# Autodesk Inventor assembly: Bunnybot
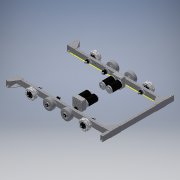
[picture p0: Inventor's stored thumbnail of the model, 180x180]
Saved by Autodesk Inventor 2018 (Build 220112000, 112)
## iProperties
Created: 2018-09-05
Part Number: Bunnybot
Document SubType Name: Assembly
Designer: baoan
Author: baoan
## Documents named in this file (16)
- C:\Users\baoan\Documents\Inventor\Bunnybots\Drivetrain\Drivetrain.iam
- C:\Users\baoan\Documents\Inventor\Bunnybots\Drivetrain\Drivetrain_length.ipt
- C:\Users\baoan\Documents\Inventor\Bunnybots\Drivetrain\Drivetrain_width.ipt
- C:\Users\baoan\Documents\Inventor\Bunnybots\Drivetrain\Center Bearing Block.ipt
- C:\Users\baoan\Documents\Inventor\Bunnybots\Drivetrain\WCP_Side_Bearing_Block_Kit_217-3436.iam
- C:\Users\baoan\Documents\Inventor\Bunnybots\Drivetrain\Drivetrain_hex_shaft.ipt
- C:\Users\baoan\Documents\Inventor\Bunnybots\Drivetrain\4_Omni-Directional_Wheel_v2_276-6194.iam
- C:\Users\baoan\Documents\Inventor\Bunnybots\Drivetrain\Hole_to_hex.ipt
- C:\Users\baoan\Documents\Inventor\Bunnybots\Drivetrain\Bearing.ipt
- C:\Users\baoan\Documents\Inventor\Bunnybots\Drivetrain\Shaft_collar.ipt
- C:\Users\baoan\Documents\Inventor\Bunnybots\Drivetrain\Drivetrain_sprockets.ipt
- C:\Users\baoan\Documents\Inventor\Bunnybots\Drivetrain\Colson_wheel.ipt
- C:\Users\baoan\Documents\Inventor\Bunnybots\Cimscellaneous\217-2454-STEP-Rev2.iam
- C:\Users\baoan\Documents\Inventor\Bunnybots\Drivetrain\Gearbox_hex_shaft.ipt
- C:\Users\baoan\Documents\Inventor\Bunnybots\Drivetrain\Drivetrain_gussets.ipt
- C:\Users\baoan\Documents\Inventor\Bunnybots\Drivetrain\Drivetrain_short_front.ipt
## Components (83 placed, 15 different names)
1. Drivetrain_width:1 — Flush:10, Flush:18, Flush:33, Mate:187, Mate:188, Flush:34, Flush:36, Mate:191, Flush:42, Flush:44, Mate:194, Flush:51, Flush:52, Flush:54
2. Drivetrain_length:3 — Angle:1, Mate:159, Flush:41, Mate:192, Flush:43, Flush:48, Mate:193, Mate:194, Flush:49, Flush:50, Flush:51, Flush:52, Mate:197, Flush:58, Flush:59
3. Center Bearing Block:2 — Insert:2
4. WCP_Side_Bearing_Block_Kit_217-3436:4 [sub-assembly] — Insert:3, Insert:5
5. WCP_Side_Bearing_Block_Kit_217-3436:5 [sub-assembly] — Insert:4, Insert:6
6. WCP_Side_Bearing_Block_Kit_217-3436:6 [sub-assembly] — Mate:38, Insert:1, Mate:39
7. Drivetrain_hex_shaft:6 — Mate:40, Mate:41, Mate:48, Mate:49, Mate:50, Mate:51, Mate:53, Mate:54, Mate:70, Mate:71, Flush:10, Flush:11
8. 4_Omni-Directional_Wheel_v2_276-6194:1 [sub-assembly] — Mate:32, Mate:33, Mate:34, Mate:35, Mate:36, Mate:37
9. Hole_to_hex:1 — Mate:32, Mate:33, Mate:34, Mate:49
10. Hole_to_hex:2 — Mate:35, Mate:36, Mate:37, Mate:48, Mate:52
11. Bearing:1 — Mate:38, Mate:39, Mate:40, Mate:41
12. Bearing:2 — Insert:1, Mate:185
13. Bearing:3 — Insert:2, Mate:100, Mate:101
14. Bearing:4 — Insert:3, Mate:68, Mate:69
15. Bearing:5 — Insert:4
16. Bearing:6 — Insert:5
17. Bearing:7 — Insert:6, Mate:90, Mate:91
18. Shaft_collar:1 — Mate:50, Mate:51, Mate:52, Flush:11
19. Drivetrain_sprockets:1 — Mate:53, Mate:54
20. Drivetrain_hex_shaft:7 — Mate:68, Mate:69, Flush:8, Mate:72, Mate:73
21. 4_Omni-Directional_Wheel_v2_276-6194:2 [sub-assembly] — Flush:13
22. Hole_to_hex:3
23. Hole_to_hex:4
24. Shaft_collar:2 — Flush:8
25. Drivetrain_sprockets:2
26. Drivetrain_sprockets:3 — Mate:70, Mate:71, Flush:31, Mate:185
27. Drivetrain_sprockets:4 — Mate:72, Mate:73, Flush:14
28. Colson_wheel:1 — Mate:87, Mate:88, Mate:89, Flush:13
29. Drivetrain_hex_shaft:8 — Mate:87, Mate:88, Mate:90, Mate:91, Mate:92, Mate:93, Mate:94, Mate:95
30. Shaft_collar:3 — Mate:89
31. Drivetrain_sprockets:5 — Mate:92, Mate:93, Mate:96, Flush:14, Flush:30
32. Drivetrain_sprockets:6 — Mate:94, Mate:95, Mate:96
33. 217-2454-STEP-Rev2:1 [sub-assembly] — Mate:97, Mate:98, Mate:99, Angle:1, Mate:159
34. Gearbox_hex_shaft:1 — Mate:97, Mate:98, Mate:99, Mate:100, Mate:101, Mate:160, Mate:161, Mate:162, Mate:163, Flush:23, Mate:167, Mate:168
35. Drivetrain_length:4 — Insert:13, Mate:183, Angle:2, Mate:186, Flush:32, Mate:187, Flush:35, Flush:36, Flush:46, Mate:195, Flush:53, Flush:54, Flush:55, Mate:199, Flush:62
36. WCP_Side_Bearing_Block_Kit_217-3436:7 [sub-assembly]
37. WCP_Side_Bearing_Block_Kit_217-3436:8 [sub-assembly]
38. WCP_Side_Bearing_Block_Kit_217-3436:9 [sub-assembly]
39. Bearing:8 — Mate:184
40. Bearing:9 — Mate:130, Mate:131
41. Bearing:11
42. Bearing:12 — Mate:157, Mate:158
43. Bearing:13 — Mate:145, Mate:146
44. Bearing:14
45. Center Bearing Block:3 — Insert:13, Insert:14
46. Bearing:15 — Insert:14, Mate:181, Mate:182
47. Drivetrain_hex_shaft:9 — Mate:130, Mate:131, Flush:18
48. 4_Omni-Directional_Wheel_v2_276-6194:3 [sub-assembly]
49. Hole_to_hex:5
50. Hole_to_hex:6
51. Shaft_collar:4
52. Drivetrain_sprockets:7 — Flush:29, Mate:184
53. Drivetrain_hex_shaft:10 — Mate:145, Mate:146
54. 4_Omni-Directional_Wheel_v2_276-6194:4 [sub-assembly] — Flush:22
55. Hole_to_hex:7
56. Hole_to_hex:8
57. Shaft_collar:5
58. Drivetrain_sprockets:8 — Flush:28
59. Colson_wheel:2 — Flush:22
60. Drivetrain_hex_shaft:11 — Mate:157, Mate:158
61. Shaft_collar:6
62. Drivetrain_sprockets:9 — Flush:27, Flush:28
63. Drivetrain_sprockets:10
64. Colson_wheel:3 — Mate:160, Mate:161, Mate:164
65. Shaft_collar:7 — Mate:162, Mate:163, Flush:23, Mate:164
66. Drivetrain_sprockets:11 — Mate:166, Flush:24, Mate:167, Mate:168, Flush:30, Flush:31
67. Drivetrain_sprockets:12 — Mate:166, Flush:24
68. 217-2454-STEP-Rev2:2 [sub-assembly] — Mate:183, Angle:2
69. Gearbox_hex_shaft:2 — Mate:181, Mate:182
70. Colson_wheel:4
71. Shaft_collar:8
72. Drivetrain_sprockets:13 — Flush:27, Flush:29
73. Drivetrain_sprockets:14
74. Drivetrain_gussets:1 — Mate:186, Flush:32, Flush:33
75. Drivetrain_gussets:2 — Mate:188, Flush:34, Flush:35
76. Drivetrain_gussets:5 — Mate:191, Flush:41, Flush:42
77. Drivetrain_gussets:6 — Mate:192, Flush:43, Flush:44
78. Drivetrain_gussets:7 — Flush:46, Mate:196, Flush:56
79. Drivetrain_gussets:8 — Flush:48, Mate:197, Flush:57, Flush:58
80. Drivetrain_short_front:1 — Mate:193, Flush:49, Flush:50, Flush:57, Mate:198, Flush:60
81. Drivetrain_short_front:2 — Mate:195, Flush:53, Mate:196, Flush:55, Flush:56, Flush:61
82. Drivetrain_gussets:9 — Mate:198, Flush:59, Flush:60
83. Drivetrain_gussets:10 — Mate:199, Flush:61, Flush:62
## Relationships (217: Mate 157, Flush 45, Insert 13, Angle 2)
- [Mate]: Drivetrain_length:3 ↔ Center Bearing Block:2
- [Mate]: Drivetrain_length:3 ↔ Center Bearing Block:2
- [Mate]: Drivetrain_length:3 ↔ Center Bearing Block:2
- [Mate]: Drivetrain_length:3 ↔ WCP_Side_Bearing_Block_Kit_217-3436:4
- [Mate]: Drivetrain_length:3 ↔ WCP_Side_Bearing_Block_Kit_217-3436:4
- [Mate]: Drivetrain_length:3 ↔ WCP_Side_Bearing_Block_Kit_217-3436:4
- [Mate]: Drivetrain_length:3 ↔ WCP_Side_Bearing_Block_Kit_217-3436:5
- [Mate]: Drivetrain_length:3 ↔ WCP_Side_Bearing_Block_Kit_217-3436:5
- [Mate]: Drivetrain_length:3 ↔ WCP_Side_Bearing_Block_Kit_217-3436:5
- [Mate]: Drivetrain_length:3 ↔ WCP_Side_Bearing_Block_Kit_217-3436:6
- [Mate]: Drivetrain_length:3 ↔ WCP_Side_Bearing_Block_Kit_217-3436:6
- [Mate]: Drivetrain_length:3 ↔ WCP_Side_Bearing_Block_Kit_217-3436:6
- Mate:32: 4_Omni-Directional_Wheel_v2_276-6194:1 ↔ Hole_to_hex:1
- Mate:33: 4_Omni-Directional_Wheel_v2_276-6194:1 ↔ Hole_to_hex:1
- Mate:34: 4_Omni-Directional_Wheel_v2_276-6194:1 ↔ Hole_to_hex:1
- Mate:35: 4_Omni-Directional_Wheel_v2_276-6194:1 ↔ Hole_to_hex:2
- Mate:36: 4_Omni-Directional_Wheel_v2_276-6194:1 ↔ Hole_to_hex:2
- Mate:37: 4_Omni-Directional_Wheel_v2_276-6194:1 ↔ Hole_to_hex:2
- Mate:38: WCP_Side_Bearing_Block_Kit_217-3436:6 ↔ Bearing:1
- Insert:1: WCP_Side_Bearing_Block_Kit_217-3436:6 ↔ Bearing:2
- Mate:39: WCP_Side_Bearing_Block_Kit_217-3436:6 ↔ Bearing:1
- Insert:2: Center Bearing Block:2 ↔ Bearing:3
- Insert:3: WCP_Side_Bearing_Block_Kit_217-3436:4 ↔ Bearing:4
- Insert:4: WCP_Side_Bearing_Block_Kit_217-3436:5 ↔ Bearing:5
- Insert:5: WCP_Side_Bearing_Block_Kit_217-3436:4 ↔ Bearing:6
- Insert:6: WCP_Side_Bearing_Block_Kit_217-3436:5 ↔ Bearing:7
- Mate:40: Drivetrain_hex_shaft:6 ↔ Bearing:1
- Mate:41: Drivetrain_hex_shaft:6 ↔ Bearing:1
- Mate:48: Drivetrain_hex_shaft:6 ↔ Hole_to_hex:2
- Mate:49: Drivetrain_hex_shaft:6 ↔ Hole_to_hex:1
- Mate:50: Drivetrain_hex_shaft:6 ↔ Shaft_collar:1
- Mate:51: Drivetrain_hex_shaft:6 ↔ Shaft_collar:1
- Mate:52: Hole_to_hex:2 ↔ Shaft_collar:1
- Mate:53: Drivetrain_hex_shaft:6 ↔ Drivetrain_sprockets:1
- Mate:54: Drivetrain_hex_shaft:6 ↔ Drivetrain_sprockets:1
- [Mate]: 4_Omni-Directional_Wheel_v2_276-6194:2 ↔ Hole_to_hex:3
- [Mate]: 4_Omni-Directional_Wheel_v2_276-6194:2 ↔ Hole_to_hex:3
- [Mate]: 4_Omni-Directional_Wheel_v2_276-6194:2 ↔ Hole_to_hex:3
- [Mate]: 4_Omni-Directional_Wheel_v2_276-6194:2 ↔ Hole_to_hex:4
- [Mate]: 4_Omni-Directional_Wheel_v2_276-6194:2 ↔ Hole_to_hex:4
- [Mate]: 4_Omni-Directional_Wheel_v2_276-6194:2 ↔ Hole_to_hex:4
- [Mate]: Drivetrain_hex_shaft:7 ↔ Hole_to_hex:4
- [Mate]: Drivetrain_hex_shaft:7 ↔ Hole_to_hex:3
- [Mate]: Drivetrain_hex_shaft:7 ↔ Shaft_collar:2
- [Mate]: Drivetrain_hex_shaft:7 ↔ Shaft_collar:2
- [Mate]: Hole_to_hex:4 ↔ Shaft_collar:2
- [Mate]: Drivetrain_hex_shaft:7 ↔ Drivetrain_sprockets:2
- [Mate]: Drivetrain_hex_shaft:7 ↔ Drivetrain_sprockets:2
- Mate:68: Bearing:4 ↔ Drivetrain_hex_shaft:7
- Mate:69: Bearing:4 ↔ Drivetrain_hex_shaft:7
- Flush:8 (-3.175 mm): Drivetrain_hex_shaft:7 ↔ Shaft_collar:2
- Mate:70: Drivetrain_hex_shaft:6 ↔ Drivetrain_sprockets:3
- Mate:71: Drivetrain_hex_shaft:6 ↔ Drivetrain_sprockets:3
- Flush:10: Drivetrain_width:1 ↔ Drivetrain_hex_shaft:6
- Flush:11 (-3.175 mm): Drivetrain_hex_shaft:6 ↔ Shaft_collar:1
- Mate:72: Drivetrain_hex_shaft:7 ↔ Drivetrain_sprockets:4
- Mate:73: Drivetrain_hex_shaft:7 ↔ Drivetrain_sprockets:4
- [Mate]: Drivetrain_hex_shaft:8 ↔ Shaft_collar:3
- [Mate]: Drivetrain_hex_shaft:8 ↔ Shaft_collar:3
- [Flush] (-3.175 mm): Drivetrain_hex_shaft:8 ↔ Shaft_collar:3
- Mate:87: Colson_wheel:1 ↔ Drivetrain_hex_shaft:8
- Mate:88: Colson_wheel:1 ↔ Drivetrain_hex_shaft:8
- Mate:89: Colson_wheel:1 ↔ Shaft_collar:3
- Mate:90: Bearing:7 ↔ Drivetrain_hex_shaft:8
- Mate:91: Bearing:7 ↔ Drivetrain_hex_shaft:8
- Flush:13: 4_Omni-Directional_Wheel_v2_276-6194:2 ↔ Colson_wheel:1
- Mate:92: Drivetrain_hex_shaft:8 ↔ Drivetrain_sprockets:5
- Mate:93: Drivetrain_hex_shaft:8 ↔ Drivetrain_sprockets:5
- Mate:94: Drivetrain_hex_shaft:8 ↔ Drivetrain_sprockets:6
- Mate:95: Drivetrain_hex_shaft:8 ↔ Drivetrain_sprockets:6
- Mate:96: Drivetrain_sprockets:5 ↔ Drivetrain_sprockets:6
- Flush:14: Drivetrain_sprockets:4 ↔ Drivetrain_sprockets:5
- Mate:97: 217-2454-STEP-Rev2:1 ↔ Gearbox_hex_shaft:1
- Mate:98: 217-2454-STEP-Rev2:1 ↔ Gearbox_hex_shaft:1
- Mate:99: 217-2454-STEP-Rev2:1 ↔ Gearbox_hex_shaft:1
- Mate:100: Bearing:3 ↔ Gearbox_hex_shaft:1
- Mate:101: Bearing:3 ↔ Gearbox_hex_shaft:1
- Angle:1 (0 deg): Drivetrain_length:3 ↔ 217-2454-STEP-Rev2:1
- [Mate]: Drivetrain_length:4 ↔ WCP_Side_Bearing_Block_Kit_217-3436:7
- [Mate]: Drivetrain_length:4 ↔ WCP_Side_Bearing_Block_Kit_217-3436:7
- [Mate]: Drivetrain_length:4 ↔ WCP_Side_Bearing_Block_Kit_217-3436:7
- [Mate]: Drivetrain_length:4 ↔ WCP_Side_Bearing_Block_Kit_217-3436:8
- [Mate]: Drivetrain_length:4 ↔ WCP_Side_Bearing_Block_Kit_217-3436:8
- [Mate]: Drivetrain_length:4 ↔ WCP_Side_Bearing_Block_Kit_217-3436:8
- [Mate]: Drivetrain_length:4 ↔ WCP_Side_Bearing_Block_Kit_217-3436:9
- [Mate]: Drivetrain_length:4 ↔ WCP_Side_Bearing_Block_Kit_217-3436:9
- [Mate]: Drivetrain_length:4 ↔ WCP_Side_Bearing_Block_Kit_217-3436:9
- [Mate]: WCP_Side_Bearing_Block_Kit_217-3436:9 ↔ Bearing:8
- [Insert]: WCP_Side_Bearing_Block_Kit_217-3436:9 ↔ Bearing:9
- [Mate]: WCP_Side_Bearing_Block_Kit_217-3436:9 ↔ Bearing:8
- [Insert]: WCP_Side_Bearing_Block_Kit_217-3436:7 ↔ Bearing:11
- [Insert]: WCP_Side_Bearing_Block_Kit_217-3436:8 ↔ Bearing:12
- [Insert]: WCP_Side_Bearing_Block_Kit_217-3436:7 ↔ Bearing:13
- [Insert]: WCP_Side_Bearing_Block_Kit_217-3436:8 ↔ Bearing:14
- Insert:13: Drivetrain_length:4 ↔ Center Bearing Block:3
- Insert:14: Center Bearing Block:3 ↔ Bearing:15
- [Mate]: 4_Omni-Directional_Wheel_v2_276-6194:3 ↔ Hole_to_hex:5
- [Mate]: 4_Omni-Directional_Wheel_v2_276-6194:3 ↔ Hole_to_hex:5
- [Mate]: 4_Omni-Directional_Wheel_v2_276-6194:3 ↔ Hole_to_hex:5
- [Mate]: 4_Omni-Directional_Wheel_v2_276-6194:3 ↔ Hole_to_hex:6
- [Mate]: 4_Omni-Directional_Wheel_v2_276-6194:3 ↔ Hole_to_hex:6
- [Mate]: 4_Omni-Directional_Wheel_v2_276-6194:3 ↔ Hole_to_hex:6
- [Mate]: Drivetrain_hex_shaft:9 ↔ Hole_to_hex:6
- [Mate]: Drivetrain_hex_shaft:9 ↔ Hole_to_hex:5
- [Mate]: Drivetrain_hex_shaft:9 ↔ Shaft_collar:4
- [Mate]: Drivetrain_hex_shaft:9 ↔ Shaft_collar:4
- [Mate]: Hole_to_hex:6 ↔ Shaft_collar:4
- [Mate]: Drivetrain_hex_shaft:9 ↔ Drivetrain_sprockets:7
- [Mate]: Drivetrain_hex_shaft:9 ↔ Drivetrain_sprockets:7
- [Flush] (-3.175 mm): Drivetrain_hex_shaft:9 ↔ Shaft_collar:4
- Mate:130: Bearing:9 ↔ Drivetrain_hex_shaft:9
- Mate:131: Bearing:9 ↔ Drivetrain_hex_shaft:9
- Flush:18: Drivetrain_width:1 ↔ Drivetrain_hex_shaft:9
- [Mate]: 4_Omni-Directional_Wheel_v2_276-6194:4 ↔ Hole_to_hex:7
- [Mate]: 4_Omni-Directional_Wheel_v2_276-6194:4 ↔ Hole_to_hex:7
- [Mate]: 4_Omni-Directional_Wheel_v2_276-6194:4 ↔ Hole_to_hex:7
- [Mate]: 4_Omni-Directional_Wheel_v2_276-6194:4 ↔ Hole_to_hex:8
- [Mate]: 4_Omni-Directional_Wheel_v2_276-6194:4 ↔ Hole_to_hex:8
- [Mate]: 4_Omni-Directional_Wheel_v2_276-6194:4 ↔ Hole_to_hex:8
- [Mate]: Drivetrain_hex_shaft:10 ↔ Hole_to_hex:8
- [Mate]: Drivetrain_hex_shaft:10 ↔ Hole_to_hex:7
- [Mate]: Drivetrain_hex_shaft:10 ↔ Shaft_collar:5
- [Mate]: Drivetrain_hex_shaft:10 ↔ Shaft_collar:5
- [Mate]: Hole_to_hex:8 ↔ Shaft_collar:5
- [Mate]: Drivetrain_hex_shaft:10 ↔ Drivetrain_sprockets:8
- [Mate]: Drivetrain_hex_shaft:10 ↔ Drivetrain_sprockets:8
- [Flush] (-3.175 mm): Drivetrain_hex_shaft:10 ↔ Shaft_collar:5
- Mate:145: Bearing:13 ↔ Drivetrain_hex_shaft:10
- Mate:146: Bearing:13 ↔ Drivetrain_hex_shaft:10
- [Mate]: Drivetrain_hex_shaft:11 ↔ Shaft_collar:6
- [Mate]: Drivetrain_hex_shaft:11 ↔ Shaft_collar:6
- [Flush] (-3.175 mm): Drivetrain_hex_shaft:11 ↔ Shaft_collar:6
- [Mate]: Colson_wheel:2 ↔ Drivetrain_hex_shaft:11
- [Mate]: Colson_wheel:2 ↔ Drivetrain_hex_shaft:11
- [Mate]: Colson_wheel:2 ↔ Shaft_collar:6
- [Mate]: Drivetrain_hex_shaft:11 ↔ Drivetrain_sprockets:9
- [Mate]: Drivetrain_hex_shaft:11 ↔ Drivetrain_sprockets:9
- [Mate]: Drivetrain_hex_shaft:11 ↔ Drivetrain_sprockets:10
- [Mate]: Drivetrain_hex_shaft:11 ↔ Drivetrain_sprockets:10
- [Mate]: Drivetrain_sprockets:9 ↔ Drivetrain_sprockets:10
- Mate:157: Bearing:12 ↔ Drivetrain_hex_shaft:11
- Mate:158: Bearing:12 ↔ Drivetrain_hex_shaft:11
- Flush:22: 4_Omni-Directional_Wheel_v2_276-6194:4 ↔ Colson_wheel:2
- Mate:159 (38.1 mm): Drivetrain_length:3 ↔ 217-2454-STEP-Rev2:1
- Mate:160: Gearbox_hex_shaft:1 ↔ Colson_wheel:3
- Mate:161: Gearbox_hex_shaft:1 ↔ Colson_wheel:3
- Mate:162: Gearbox_hex_shaft:1 ↔ Shaft_collar:7
- Mate:163: Gearbox_hex_shaft:1 ↔ Shaft_collar:7
- Flush:23 (-3.175 mm): Gearbox_hex_shaft:1 ↔ Shaft_collar:7
- Mate:164: Colson_wheel:3 ↔ Shaft_collar:7
- [Mate]: Drivetrain_sprockets:11 ↔ Drivetrain_sprockets:12
- Mate:166: Drivetrain_sprockets:11 ↔ Drivetrain_sprockets:12
- Flush:24: Drivetrain_sprockets:11 ↔ Drivetrain_sprockets:12
- Mate:167: Gearbox_hex_shaft:1 ↔ Drivetrain_sprockets:11
- Mate:168: Gearbox_hex_shaft:1 ↔ Drivetrain_sprockets:11
- [Mate]: 217-2454-STEP-Rev2:2 ↔ Gearbox_hex_shaft:2
- [Mate]: 217-2454-STEP-Rev2:2 ↔ Gearbox_hex_shaft:2
- [Mate]: 217-2454-STEP-Rev2:2 ↔ Gearbox_hex_shaft:2
- [Mate]: Gearbox_hex_shaft:2 ↔ Colson_wheel:4
- [Mate]: Gearbox_hex_shaft:2 ↔ Colson_wheel:4
- [Mate]: Gearbox_hex_shaft:2 ↔ Shaft_collar:8
- [Mate]: Gearbox_hex_shaft:2 ↔ Shaft_collar:8
- [Flush] (-3.175 mm): Gearbox_hex_shaft:2 ↔ Shaft_collar:8
- [Mate]: Colson_wheel:4 ↔ Shaft_collar:8
- [Mate]: Drivetrain_sprockets:13 ↔ Drivetrain_sprockets:14
- [Mate]: Drivetrain_sprockets:13 ↔ Drivetrain_sprockets:14
- [Flush]: Drivetrain_sprockets:13 ↔ Drivetrain_sprockets:14
- [Mate]: Gearbox_hex_shaft:2 ↔ Drivetrain_sprockets:13
- [Mate]: Gearbox_hex_shaft:2 ↔ Drivetrain_sprockets:13
- Mate:181: Bearing:15 ↔ Gearbox_hex_shaft:2
- Mate:182: Bearing:15 ↔ Gearbox_hex_shaft:2
- Mate:183 (38.1 mm): Drivetrain_length:4 ↔ 217-2454-STEP-Rev2:2
- Flush:27: Drivetrain_sprockets:9 ↔ Drivetrain_sprockets:13
- Flush:28: Drivetrain_sprockets:8 ↔ Drivetrain_sprockets:9
- Flush:29: Drivetrain_sprockets:7 ↔ Drivetrain_sprockets:13
- Flush:30: Drivetrain_sprockets:5 ↔ Drivetrain_sprockets:11
- Flush:31: Drivetrain_sprockets:3 ↔ Drivetrain_sprockets:11
- Mate:184 (8.255 mm): Bearing:8 ↔ Drivetrain_sprockets:7
- Mate:185 (8.255 mm): Bearing:2 ↔ Drivetrain_sprockets:3
- Angle:2 (0 deg): Drivetrain_length:4 ↔ 217-2454-STEP-Rev2:2
- Mate:186: Drivetrain_length:4 ↔ Drivetrain_gussets:1
- Flush:32: Drivetrain_length:4 ↔ Drivetrain_gussets:1
- Flush:33: Drivetrain_width:1 ↔ Drivetrain_gussets:1
- Mate:187: Drivetrain_width:1 ↔ Drivetrain_length:4
- Mate:188: Drivetrain_width:1 ↔ Drivetrain_gussets:2
- Flush:34: Drivetrain_width:1 ↔ Drivetrain_gussets:2
- Flush:35: Drivetrain_length:4 ↔ Drivetrain_gussets:2
- Flush:36: Drivetrain_width:1 ↔ Drivetrain_length:4
- Mate:191: Drivetrain_width:1 ↔ Drivetrain_gussets:5
- Flush:41: Drivetrain_length:3 ↔ Drivetrain_gussets:5
- Flush:42: Drivetrain_width:1 ↔ Drivetrain_gussets:5
- Mate:192: Drivetrain_length:3 ↔ Drivetrain_gussets:6
- Flush:43: Drivetrain_length:3 ↔ Drivetrain_gussets:6
- Flush:44: Drivetrain_width:1 ↔ Drivetrain_gussets:6
- Flush:46: Drivetrain_length:4 ↔ Drivetrain_gussets:7
- Flush:48: Drivetrain_length:3 ↔ Drivetrain_gussets:8
- Mate:193: Drivetrain_length:3 ↔ Drivetrain_short_front:1
- Mate:194: Drivetrain_width:1 ↔ Drivetrain_length:3
- Flush:49: Drivetrain_length:3 ↔ Drivetrain_short_front:1
- Flush:50: Drivetrain_length:3 ↔ Drivetrain_short_front:1
- Flush:51 (76.2 mm): Drivetrain_width:1 ↔ Drivetrain_length:3
- Flush:52: Drivetrain_width:1 ↔ Drivetrain_length:3
- Mate:195: Drivetrain_length:4 ↔ Drivetrain_short_front:2
- Flush:53: Drivetrain_length:4 ↔ Drivetrain_short_front:2
- Mate:196: Drivetrain_gussets:7 ↔ Drivetrain_short_front:2
- Flush:54 (76.2 mm): Drivetrain_width:1 ↔ Drivetrain_length:4
- Flush:55: Drivetrain_length:4 ↔ Drivetrain_short_front:2
- Flush:56: Drivetrain_gussets:7 ↔ Drivetrain_short_front:2
- Mate:197: Drivetrain_length:3 ↔ Drivetrain_gussets:8
- Flush:57: Drivetrain_gussets:8 ↔ Drivetrain_short_front:1
- Flush:58: Drivetrain_length:3 ↔ Drivetrain_gussets:8
- Mate:198: Drivetrain_short_front:1 ↔ Drivetrain_gussets:9
- Flush:59: Drivetrain_length:3 ↔ Drivetrain_gussets:9
- Flush:60: Drivetrain_short_front:1 ↔ Drivetrain_gussets:9
- Mate:199: Drivetrain_length:4 ↔ Drivetrain_gussets:10
- Flush:61: Drivetrain_short_front:2 ↔ Drivetrain_gussets:10
- Flush:62: Drivetrain_length:4 ↔ Drivetrain_gussets:10
## Named parameters: d33_d18 = 0 mm, d34_d19 = 0 mm, d35_d22 = 0 mm, d36_d24 = 0 mm, d37_d25 = 0 mm, d38_d26 = 0 mm, d39_d27 = 0 mm, d40_d28 = 0 mm, d41_d29 = 0 mm, d42_d30 = 0 mm, d43_d31 = 0 mm, d44_d32 = 0 mm, d78_d71 = 0 mm, d79_d72 = 0 mm, d80_d73 = 0 mm, d81_d74 = 0 mm, d82_d75 = 0 mm, d83_d76 = 0 mm, d84_d77 = 0 mm, d85_d48 = 0 mm, d86_d49 = 0 mm, d87_d50 = 0 mm, d88_d51 = 0 mm, d89_d52 = 0 mm, d90_d53 = 0 mm, d105_d80_d73 = 0 mm, d106_d81_d74 = 0 mm, d114_d93 = -3.175 mm, d139_d36_d24 = 0 mm, d140_d37_d25 = 0 mm, d141_d38_d26 = 0 mm, d142_d39_d27 = 0 mm, d143_d40_d28 = 0 mm, d144_d41_d29 = 0 mm, d145_d42_d30 = 0 mm, d146_d43_d31 = 0 mm, d147_d44_d32 = 0 mm, d148_d54 = 0 mm, d149_d56 = 0 mm, d150_d57 = 0 mm, d152_d59 = 0 mm, d153_d60 = 0 mm, d154_d61 = 0 mm, d155_d62 = 0 mm, d161_d98 = -3.175 mm, d162_d71 = 0 mm, d163_d72 = 0 mm, d164_d73 = 0 mm, d165_d74 = 0 mm, d166_d75 = 0 mm, d167_d95 = 0 mm, d168_d96 = 0 mm, d169_d48 = 0 mm, d170_d49 = 0 mm, d171_d50 = 0 mm, d172_d51 = 0 mm, d173_d52 = 0 mm, d174_d53 = 0 mm, d178_d161_d98 = -3.175 mm, d179_d162_d71 = 0 mm, d180_d163_d72 = 0 mm, d181_d164_d73 = 0 mm, d182_d165_d74 = 0 mm, d183_d166_d75 = 0 mm, d184_d167_d95 = 0 mm, d185_d168_d96 = 0 mm, d186_d169_d48 = 0 mm, d187_d170_d49 = 0 mm, d188_d171_d50 = 0 mm, d189_d172_d51 = 0 mm, d190_d173_d52 = 0 mm, d191_d174_d53 = 0 mm, d195_d124 = 0 mm, d196_d125 = 0 mm, d197_d105_d80_d73 = 0 mm, d198_d106_d81_d74 = 0 mm, d199_d114_d93 = -3.175 mm, d200_d115 = 0 mm, d201_d116 = 0 mm, d202_d117 = 0 mm, d203_d121 = 0 mm, d204_d122 = 0 mm, d205_d123 = 0 mm, d216_d125 = 0 mm, d221_d214 = -3.175 mm, d222_d215 = 0 mm, d223_d216_d125 = 0 mm, d224_d217 = 0 mm, d225_d218 = 0 mm, d226_d219 = 0 mm, d227_d220 = 0 mm, d228_d210 = 0 mm, d229_d211 = 0 mm, d230_d212 = 0 mm, d231_d213 = 0 mm, d232_d127 = 0 mm, d233_d128 = 0 mm, d234_d129 = 0 mm
